# Autodesk Inventor assembly: FullWheelAJB
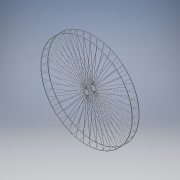
[picture p0: Inventor's stored thumbnail of the model, 180x180]
Saved by Autodesk Inventor 2018 (Build 220112000, 112)
## iProperties
Created: 2018-01-18
Part Number: FullWheelAJB
Document SubType Name: Assembly
Designer: Alec temporary
Author: Alec temporary
## Documents named in this file (3)
- C:\Users\Alec temporary\Desktop\New folder\FullWheelAJB.iam
- C:\Users\Alec temporary\Desktop\New folder\HalfWheelAJB.iam
- C:\Users\Alec temporary\Desktop\New folder\ConnectionBarAJB.ipt
## Components (42 placed, 2 different names)
1. HalfWheelAJB:1 [sub-assembly] — Mate:1, Flush:1, Mate:2
2. HalfWheelAJB:2 [sub-assembly] — Mate:2, Mate:3, Flush:2
3. ConnectionBarAJB:1 — Mate:1, Flush:1, Mate:3, Flush:2
4. ConnectionBarAJB:2
5. ConnectionBarAJB:3
6. ConnectionBarAJB:4
7. ConnectionBarAJB:5
8. ConnectionBarAJB:6
9. ConnectionBarAJB:7
10. ConnectionBarAJB:8
11. ConnectionBarAJB:9
12. ConnectionBarAJB:10
13. ConnectionBarAJB:11
14. ConnectionBarAJB:12
15. ConnectionBarAJB:13
16. ConnectionBarAJB:14
17. ConnectionBarAJB:15
18. ConnectionBarAJB:16
19. ConnectionBarAJB:17
20. ConnectionBarAJB:18
21. ConnectionBarAJB:19
22. ConnectionBarAJB:20
23. ConnectionBarAJB:21
24. ConnectionBarAJB:22
25. ConnectionBarAJB:23
26. ConnectionBarAJB:24
27. ConnectionBarAJB:25
28. ConnectionBarAJB:26
29. ConnectionBarAJB:27
30. ConnectionBarAJB:28
31. ConnectionBarAJB:29
32. ConnectionBarAJB:30
33. ConnectionBarAJB:31
34. ConnectionBarAJB:32
35. ConnectionBarAJB:33
36. ConnectionBarAJB:34
37. ConnectionBarAJB:35
38. ConnectionBarAJB:36
39. ConnectionBarAJB:37
40. ConnectionBarAJB:38
41. ConnectionBarAJB:39
42. ConnectionBarAJB:40
## Component patterns: (40 elements, first: ConnectionBarAJB:1)
## Relationships (5: Mate 3, Flush 2)
- Mate:1: HalfWheelAJB:1 ↔ ConnectionBarAJB:1
- Flush:1: HalfWheelAJB:1 ↔ ConnectionBarAJB:1
- Mate:2: HalfWheelAJB:1 ↔ HalfWheelAJB:2
- Mate:3: HalfWheelAJB:2 ↔ ConnectionBarAJB:1
- Flush:2: HalfWheelAJB:2 ↔ ConnectionBarAJB:1
